# Autodesk Inventor assembly: Impedance_Analyzer_V2
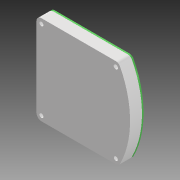
[picture p0: Inventor's stored thumbnail of the model, 180x180]
Saved by Autodesk Inventor 2021 (Build 250183000, 183)
## iProperties
Company: Kicad
Created: 2022-08-24
Part Number: Impedance_Analyzer_V2
Description: KiCad electronic assembly
Document SubType Name: Assembly
Designer: Eli
Authority: Unknown
Title: Impedance_Analyzer_V2.step
Author: Pcbnew
Sending System: KiCad to STEP converter
Preprocessor: Open CASCADE STEP processor 7.5
## Documents named in this file (3)
- C:\Users\Eli\Documents\GitHub\Simple_Impedance_Analyzer\Impedance_Analyzer_V2_KiCAD\Impedance_Analyzer_V2.iam
- C:\Users\Eli\Documents\GitHub\Simple_Impedance_Analyzer\Impedance_Analyzer_V2_KiCAD\Impedance_Analyzer_V2 PCB.ipt
- C:\Users\Eli\Documents\GitHub\Simple_Impedance_Analyzer\3D print case\Bottom Case.ipt
## Components (2 placed, 2 different names)
1. 1 — Flush:1
2. Bottom Case:1 — Flush:1
## Relationships (1: Flush 1)
- Flush:1: 1 ↔ Bottom Case:1
